# Autodesk Inventor assembly: CIM_MotorHub_4_inch_wheel_MIR
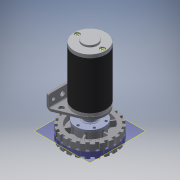
[picture p0: Inventor's stored thumbnail of the model, 180x180]
Saved by Autodesk Inventor 2016 SP1 (Build 200210100, 210)
## iProperties
Created: 2016-02-07
Part Number: CIM_MotorHub_4_inch_wheel_MIR
Document SubType Name: Assembly
Designer: steele
Author: steele
## Documents named in this file (5)
- C:\snobotics\CAD-Development\robSteele\SnoBotics2016\2016-05-05-ShooterPrototype\CIM_MotorHub_4_inch_wheel_MIR.iam
- C:\snobotics\CAD-Development\robSteele\SnoBotics2016\AM Parts\4 in HiGrip Wheel_MIR1.iam
- C:\snobotics\CAD-Development\robSteele\SnoBotics2016\AM Parts\am-0320a_8mm_Key_Hub_MIR.ipt
- C:\snobotics\CAD-Development\robSteele\SnoBotics2016\AM Parts\MOT_CIM-Motor_217-2000_MIR2.iam
- C:\snobotics\CAD-Development\robSteele\SnoBotics2016\AM Parts\AM 2488 CIM bracket_MIR.ipt
## Components (4 placed, 4 different names)
1. 4 in HiGrip Wheel_MIR1:1 [sub-assembly] — Insert:1
2. am-0320a_8mm_Key_Hub_MIR:1 — Insert:1, Insert:3
3. MOT_CIM-Motor_217-2000_MIR2:1 [sub-assembly] — Insert:2
4. AM 2488 CIM bracket_MIR:1 — Insert:3, Insert:2
## Relationships (3: Insert 3)
- Insert:1: 4 in HiGrip Wheel_MIR1:1 ↔ am-0320a_8mm_Key_Hub_MIR:1
- Insert:3: am-0320a_8mm_Key_Hub_MIR:1 ↔ AM 2488 CIM bracket_MIR:1
- Insert:2: MOT_CIM-Motor_217-2000_MIR2:1 ↔ AM 2488 CIM bracket_MIR:1
